# Autodesk Inventor assembly: Assembly SERVO
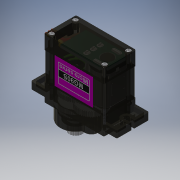
[picture p0: Inventor's stored thumbnail of the model, 180x180]
Saved by Autodesk Inventor 2019 (Build 230136000, 136)
## iProperties
Created: 2021-01-21
Part Number: Assembly SERVO
Document SubType Name: Assembly
Designer: CS
Author: CS
## Documents named in this file (4)
- C:\Users\caspe\OneDrive\Documenten\Inventor\servo\inventor files2\Assembly SERVO.iam
- C:\Users\caspe\OneDrive\Documenten\Inventor\servo\Assembly servo inside.ipt
- C:\Users\caspe\OneDrive\Documenten\Inventor\servo\Assembly servo outside.ipt
- C:\Users\caspe\Downloads\20210119_143510.jpg
## Components (2 placed, 2 different names)
1. Assembly servo inside:1 — Insert:1, Flush:1, Flush:2
2. Assembly servo outside:1 — Insert:1
## Relationships (3: Flush 2, Insert 1)
- Insert:1: Assembly servo inside:1 ↔ Assembly servo outside:1
- Flush:1: Assembly servo inside:1
- Flush:2: Assembly servo inside:1
